# Autodesk Inventor assembly: Fixture Assembly
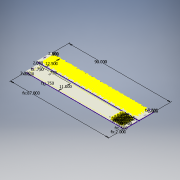
[picture p0: Inventor's stored thumbnail of the model, 180x180]
Saved by Autodesk Inventor 2018 (Build 220112000, 112)
## iProperties
Created: 2016-04-08
Part Number: Fixture Assembly
Document SubType Name: Assembly
Designer: Sam Clay
Author: Sam Clay
## Documents named in this file (6)
- Z:\enclosure\inventor\Fixture Assembly.iam
- Z:\enclosure\inventor\Fixture Base.ipt
- Z:\enclosure\inventor\Case Top Contour Fixture.ipt
- Z:\enclosure\inventor\Case Bottom Contour Fixture.ipt
- Z:\enclosure\inventor\Case Top Pocket Fixture.ipt
- Z:\enclosure\inventor\Case Bottom Pocket Fixture.ipt
## Components (145 placed, 5 different names)
1. Fixture Base:1 — Mate:27, Mate:28, Mate:35, Mate:36, Mate:38, Mate:40
2. Case Top Pocket Fixture:1 — Mate:34, Mate:35, Mate:36, Mate:39
3. Case Bottom Pocket Fixture:1 — Mate:34, Mate:38, Mate:39
4. Case Top Pocket Fixture:3
5. Case Bottom Pocket Fixture:2
6. Case Top Pocket Fixture:4
7. Case Bottom Pocket Fixture:3
8. Case Top Pocket Fixture:5
9. Case Bottom Pocket Fixture:4
10. Case Top Pocket Fixture:6
11. Case Bottom Pocket Fixture:5
12. Case Top Pocket Fixture:7
13. Case Bottom Pocket Fixture:6
14. Case Top Pocket Fixture:50
15. Case Bottom Pocket Fixture:49
16. Case Top Pocket Fixture:51
17. Case Bottom Pocket Fixture:50
18. Case Top Pocket Fixture:52
19. Case Bottom Pocket Fixture:51
20. Case Top Pocket Fixture:53
21. Case Bottom Pocket Fixture:52
22. Case Top Pocket Fixture:54
23. Case Bottom Pocket Fixture:53
24. Case Top Pocket Fixture:55
25. Case Bottom Pocket Fixture:54
26. Case Top Pocket Fixture:56
27. Case Bottom Pocket Fixture:55
28. Case Top Pocket Fixture:57
29. Case Bottom Pocket Fixture:56
30. Case Top Pocket Fixture:58
31. Case Bottom Pocket Fixture:57
32. Case Top Pocket Fixture:59
33. Case Bottom Pocket Fixture:58
34. Case Top Pocket Fixture:60
35. Case Bottom Pocket Fixture:59
36. Case Top Pocket Fixture:61
37. Case Bottom Pocket Fixture:60
38. Case Top Pocket Fixture:62
39. Case Bottom Pocket Fixture:61
40. Case Top Pocket Fixture:63
41. Case Bottom Pocket Fixture:62
42. Case Top Pocket Fixture:64
43. Case Bottom Pocket Fixture:63
44. Case Top Pocket Fixture:65
45. Case Bottom Pocket Fixture:64
46. Case Top Pocket Fixture:66
47. Case Bottom Pocket Fixture:65
48. Case Top Pocket Fixture:67
49. Case Bottom Pocket Fixture:66
50. Case Top Pocket Fixture:68
51. Case Bottom Pocket Fixture:67
52. Case Top Pocket Fixture:69
53. Case Bottom Pocket Fixture:68
54. Case Top Pocket Fixture:70
55. Case Bottom Pocket Fixture:69
56. Case Top Pocket Fixture:71
57. Case Bottom Pocket Fixture:70
58. Case Top Pocket Fixture:72
59. Case Bottom Pocket Fixture:71
60. Case Top Pocket Fixture:73
61. Case Bottom Pocket Fixture:72
62. Case Top Pocket Fixture:74
63. Case Bottom Pocket Fixture:73
64. Case Top Pocket Fixture:75
65. Case Bottom Pocket Fixture:74
66. Case Top Pocket Fixture:76
67. Case Bottom Pocket Fixture:75
68. Case Top Pocket Fixture:77
69. Case Bottom Pocket Fixture:76
70. Case Top Pocket Fixture:78
71. Case Bottom Pocket Fixture:77
72. Case Top Pocket Fixture:79
73. Case Bottom Pocket Fixture:78
74. Case Top Pocket Fixture:80
75. Case Bottom Pocket Fixture:79
76. Case Top Pocket Fixture:81
77. Case Bottom Pocket Fixture:80
78. Case Top Pocket Fixture:82
79. Case Bottom Pocket Fixture:81
80. Case Top Pocket Fixture:83
81. Case Bottom Pocket Fixture:82
82. Case Top Pocket Fixture:84
83. Case Bottom Pocket Fixture:83
84. Case Top Pocket Fixture:85
85. Case Bottom Pocket Fixture:84
86. Case Top Pocket Fixture:86
87. Case Bottom Pocket Fixture:85
88. Case Top Pocket Fixture:87
89. Case Bottom Pocket Fixture:86
90. Case Top Pocket Fixture:88
91. Case Bottom Pocket Fixture:87
92. Case Top Pocket Fixture:89
93. Case Bottom Pocket Fixture:88
94. Case Top Pocket Fixture:90
95. Case Bottom Pocket Fixture:89
96. Case Top Pocket Fixture:91
97. Case Bottom Pocket Fixture:90
98. Case Top Pocket Fixture:92
99. Case Bottom Pocket Fixture:91
100. Case Top Pocket Fixture:93
101. Case Bottom Pocket Fixture:92
102. Case Top Pocket Fixture:94
103. Case Bottom Pocket Fixture:93
104. Case Top Pocket Fixture:95
105. Case Bottom Pocket Fixture:94
106. Case Top Pocket Fixture:96
107. Case Bottom Pocket Fixture:95
108. Case Top Pocket Fixture:97
109. Case Bottom Pocket Fixture:96
110. Case Top Pocket Fixture:98
111. Case Bottom Pocket Fixture:97
112. Case Top Pocket Fixture:99
113. Case Bottom Pocket Fixture:98
114. Case Top Pocket Fixture:100
115. Case Bottom Pocket Fixture:99
116. Case Top Pocket Fixture:101
117. Case Bottom Pocket Fixture:100
118. Case Top Pocket Fixture:102
119. Case Bottom Pocket Fixture:101
120. Case Top Pocket Fixture:103
121. Case Bottom Pocket Fixture:102
122. Case Top Pocket Fixture:104
123. Case Bottom Pocket Fixture:103
124. Case Top Pocket Fixture:105
125. Case Bottom Pocket Fixture:104
126. Case Top Pocket Fixture:106
127. Case Bottom Pocket Fixture:105
128. Case Top Pocket Fixture:107
129. Case Bottom Pocket Fixture:106
130. Case Top Contour Fixture:1 — Mate:27, Mate:28, Mate:31, Mate:32, Mate:40
131. Case Bottom Contour Fixture:16 — Mate:31, Mate:32
132. Case Top Contour Fixture:2
133. Case Bottom Contour Fixture:17
134. Case Top Contour Fixture:3
135. Case Bottom Contour Fixture:18
136. Case Top Contour Fixture:4
137. Case Bottom Contour Fixture:19
138. Case Top Contour Fixture:5
139. Case Bottom Contour Fixture:20
140. Case Top Contour Fixture:6
141. Case Bottom Contour Fixture:21
142. Case Top Contour Fixture:7
143. Case Bottom Contour Fixture:22
144. Case Top Contour Fixture:8
145. Case Bottom Contour Fixture:23
## Component patterns: (8 elements), (1 elements), (8 elements, first: Case Top Pocket Fixture:1 + Case Bottom Pocket Fixture:1), Component Pattern 10:2 (8 elements), Component Pattern 10:3 (8 elements), Component Pattern 10:4 (8 elements), Component Pattern 10:5 (8 elements), Component Pattern 10:6 (8 elements), Component Pattern 10:7 (8 elements), Component Pattern 10:8 (8 elements), (8 elements, first: Case Top Contour Fixture:1 + Case Bottom Contour Fixture:16)
## Relationships (10: Mate 10)
- Mate:27 (25.4 mm): Fixture Base:1 ↔ Case Top Contour Fixture:1
- Mate:28 (35.56 mm): Fixture Base:1 ↔ Case Top Contour Fixture:1
- Mate:31: Case Top Contour Fixture:1 ↔ Case Bottom Contour Fixture:16
- Mate:32 (7.8994 mm): Case Top Contour Fixture:1 ↔ Case Bottom Contour Fixture:16
- Mate:34: Case Top Pocket Fixture:1 ↔ Case Bottom Pocket Fixture:1
- Mate:35 (19.05 mm): Fixture Base:1 ↔ Case Top Pocket Fixture:1
- Mate:36 (3.175 mm): Fixture Base:1 ↔ Case Top Pocket Fixture:1
- Mate:38: Fixture Base:1 ↔ Case Bottom Pocket Fixture:1
- Mate:39 (7.8994 mm): Case Top Pocket Fixture:1 ↔ Case Bottom Pocket Fixture:1
- Mate:40 (17.78 mm): Fixture Base:1 ↔ Case Top Contour Fixture:1
